# Autodesk Inventor assembly: assembl nozzle
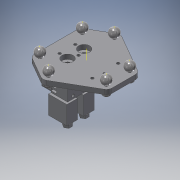
[picture p0: Inventor's stored thumbnail of the model, 180x180]
Saved by Autodesk Inventor 2016 SP1 (Build 200210100, 210)
## iProperties
Created: 2016-04-15
Part Number: assembl nozzle
Document SubType Name: Assembly
Designer: ubik
Author: ubik
## Documents named in this file (9)
- E:\GitHub\kossel-XXL\assembl nozzle.iam
- E:\GitHub\kossel-XXL\efector.ipt
- E:\GitHub\kossel-XXL\nozzel heat sink.ipt
- E:\GitHub\kossel-XXL\nozzle throat.ipt
- E:\GitHub\kossel-XXL\30x30 fan cooler.ipt
- C:\Users\ubik\Documents\Inventor\Content Center Files\R2016\en-US\AS 1420\AS 1420 - 1973 - M4 x 8.ipt
- E:\GitHub\kossel-XXL\10mm sfere.ipt
- E:\GitHub\kossel-XXL\heated block.ipt
- E:\GitHub\kossel-XXL\nozzle.ipt
## Components (21 placed, 8 different names)
1. efector:1 — Mate:5, Mate:6, Mate:7, Insert:1, Insert:2, Insert:3, Insert:4, Insert:5, Insert:6, Tangent:1
2. nozzel heat sink:1 — Mate:1, Mate:2, Mate:3, Mate:4, Mate:5, Mate:6, Mate:7, Mate:8, Flush:1, Flush:2, Mate:12
3. nozzle throat:1 — Mate:1, Mate:3, Mate:10
4. nozzle throat:2 — Mate:2, Mate:4, Mate:11
5. 30x30 fan cooler:1 — Mate:8, Flush:1, Flush:2
6. heated block:1 — Mate:10, Flush:3, Mate:12, Mate:13, Mate:15
7. heated block:2 — Mate:11, Flush:3, Mate:14
8. nozzle:1 — Mate:13, Flush:4, Mate:15
9. nozzle:2 — Mate:14, Flush:4
10. AS 1420 - Metric M4 x 8:1 — Insert:1
11. AS 1420 - Metric M4 x 8:2 — Insert:2
12. AS 1420 - Metric M4 x 8:3 — Insert:3, Mate:9
13. AS 1420 - Metric M4 x 8:4 — Insert:4
14. AS 1420 - Metric M4 x 8:5 — Insert:5
15. AS 1420 - Metric M4 x 8:6 — Insert:6
16. 10mm sfere:1 — Mate:9, Tangent:1
17. 10mm sfere:2
18. 10mm sfere:3
19. 10mm sfere:4
20. 10mm sfere:5
21. 10mm sfere:6
## Component patterns: (3 elements), (2 elements, first: 10mm sfere:1), Component Pattern 1:2 (2 elements), Component Pattern 1:3 (2 elements)
## Relationships (26: Mate 15, Insert 6, Flush 4, Tangent 1)
- Mate:1: nozzel heat sink:1 ↔ nozzle throat:1
- Mate:2: nozzel heat sink:1 ↔ nozzle throat:2
- Mate:3: nozzel heat sink:1 ↔ nozzle throat:1
- Mate:4: nozzel heat sink:1 ↔ nozzle throat:2
- Mate:5: efector:1 ↔ nozzel heat sink:1
- Mate:6: efector:1 ↔ nozzel heat sink:1
- Mate:7: efector:1 ↔ nozzel heat sink:1
- Mate:8: nozzel heat sink:1 ↔ 30x30 fan cooler:1
- Flush:1: nozzel heat sink:1 ↔ 30x30 fan cooler:1
- Flush:2: nozzel heat sink:1 ↔ 30x30 fan cooler:1
- Insert:1: efector:1 ↔ AS 1420 - Metric M4 x 8:1
- Insert:2: efector:1 ↔ AS 1420 - Metric M4 x 8:2
- Insert:3: efector:1 ↔ AS 1420 - Metric M4 x 8:3
- Insert:4: efector:1 ↔ AS 1420 - Metric M4 x 8:4
- Insert:5: efector:1 ↔ AS 1420 - Metric M4 x 8:5
- Insert:6: efector:1 ↔ AS 1420 - Metric M4 x 8:6
- Mate:9: AS 1420 - Metric M4 x 8:3 ↔ 10mm sfere:1
- Tangent:1: efector:1 ↔ 10mm sfere:1
- Mate:10: nozzle throat:1 ↔ heated block:1
- Mate:11: nozzle throat:2 ↔ heated block:2
- Flush:3: heated block:1 ↔ heated block:2
- Mate:12 (3 mm): nozzel heat sink:1 ↔ heated block:1
- Mate:13: heated block:1 ↔ nozzle:1
- Mate:14: heated block:2 ↔ nozzle:2
- Flush:4: nozzle:1 ↔ nozzle:2
- Mate:15 (2 mm): heated block:1 ↔ nozzle:1
